# Autodesk Inventor assembly: 090 ASY bottom
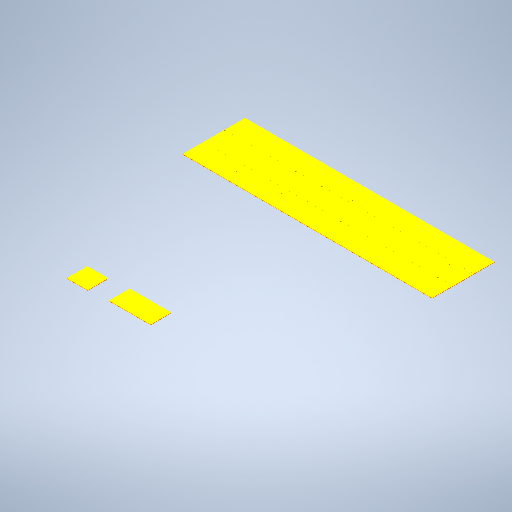
[picture p0: Inventor's stored thumbnail of the model, 512x512]
Saved by Autodesk Inventor 2026 (Build 300175000, 175)
## iProperties
Created: 2026-05-19
Part Number: 090 ASY bottom
Document SubType Name: Assembly
Designer: user
Author: user
## Documents named in this file (9)
- C:\Users\user\Documents\Inventor\GBK-Gubkinskiy\090 ASY bottom.iam
- C:\Users\user\Documents\Inventor\GBK-Gubkinskiy\0910.ipt
- C:\Users\user\Documents\Inventor\GBK-Gubkinskiy\092.iam
- C:\Users\user\Documents\Inventor\GBK-Gubkinskiy\093.iam
- C:\Users\user\Documents\Inventor\GBK-Gubkinskiy\092_CPY.iam
- C:\Users\user\Documents\Inventor\GBK-Gubkinskiy\093_CPY.iam
- C:\Users\user\Documents\Inventor\GBK-Gubkinskiy\092_CPY1.iam
- C:\Users\user\Documents\Inventor\GBK-Gubkinskiy\093_CPY1.iam
- C:\Users\user\Documents\Inventor\GBK-Gubkinskiy\092_CPY_CPY.iam
## Components (22 placed, 8 different names)
1. 0910:1 — Заподлицо:1, Заподлицо:2, Жесткий:1
2. 092:1 [sub-assembly] — Заподлицо:1
3. 093:1 [sub-assembly] — Заподлицо:2
4. 093_CPY:1 [sub-assembly] — Заподлицо:3, Заподлицо:4, Совмещение:1, Заподлицо:5, Заподлицо:6, Совмещение:2, Заподлицо:9, Заподлицо:10, Совмещение:4
5. 093_CPY1:1 [sub-assembly] — Заподлицо:7, Заподлицо:8, Совмещение:3
6. 092_CPY:1 [sub-assembly] — Жесткий:1, Заподлицо:3, Заподлицо:4, Совмещение:1
7. 092_CPY:2 [sub-assembly]
8. 092_CPY:3 [sub-assembly]
9. 092_CPY:4 [sub-assembly]
10. 092_CPY:5 [sub-assembly]
11. 092_CPY:6 [sub-assembly]
12. 092_CPY1:1 [sub-assembly] — Заподлицо:5, Заподлицо:6, Совмещение:2
13. 092_CPY1:2 [sub-assembly]
14. 092_CPY1:3 [sub-assembly]
15. 092_CPY1:4 [sub-assembly]
16. 092_CPY1:5 [sub-assembly] — Заподлицо:7, Заподлицо:8, Совмещение:3
17. 092_CPY_CPY:1 [sub-assembly] — Заподлицо:9, Заподлицо:10, Совмещение:4
18. 092_CPY_CPY:2 [sub-assembly]
19. 092_CPY_CPY:3 [sub-assembly]
20. 092_CPY_CPY:4 [sub-assembly]
21. 092_CPY_CPY:5 [sub-assembly]
22. 092_CPY_CPY:6 [sub-assembly]
## Component patterns: (6 elements, first: 092_CPY:1), (5 elements, first: 092_CPY1:1), (6 elements, first: 092_CPY_CPY:1)
## Relationships (15: Flush 10, Mate 4, WeldJoint 1)
- Заподлицо:1 [Flush]: 0910:1 ↔ 092:1
- Заподлицо:2 [Flush]: 0910:1 ↔ 093:1
- Жесткий:1 [WeldJoint]: 0910:1 ↔ 092_CPY:1
- Заподлицо:3 [Flush]: 093_CPY:1 ↔ 092_CPY:1
- Заподлицо:4 [Flush]: 093_CPY:1 ↔ 092_CPY:1
- Совмещение:1 [Mate] (4 mm): 093_CPY:1 ↔ 092_CPY:1
- Заподлицо:5 [Flush]: 093_CPY:1 ↔ 092_CPY1:1
- Заподлицо:6 [Flush]: 093_CPY:1 ↔ 092_CPY1:1
- Совмещение:2 [Mate] (4 mm): 093_CPY:1 ↔ 092_CPY1:1
- Заподлицо:7 [Flush]: 093_CPY1:1 ↔ 092_CPY1:5
- Заподлицо:8 [Flush]: 093_CPY1:1 ↔ 092_CPY1:5
- Совмещение:3 [Mate]: 093_CPY1:1 ↔ 092_CPY1:5
- Заподлицо:9 [Flush]: 093_CPY:1 ↔ 092_CPY_CPY:1
- Заподлицо:10 [Flush]: 093_CPY:1 ↔ 092_CPY_CPY:1
- Совмещение:4 [Mate]: 093_CPY:1 ↔ 092_CPY_CPY:1
